# Autodesk Inventor assembly: ASY PNS 1600 Filter column D1000
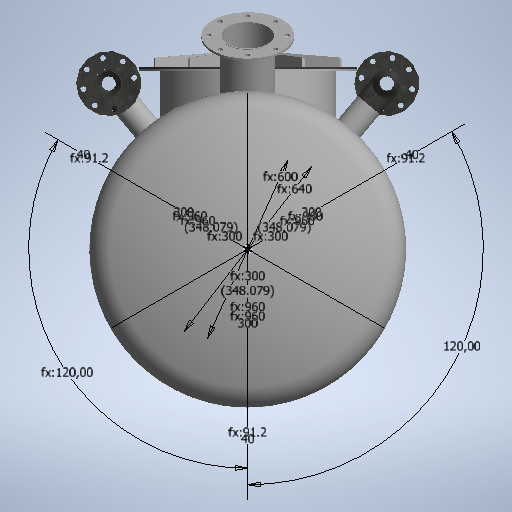
[picture p0: Inventor's stored thumbnail of the model, 512x512]
Saved by Autodesk Inventor 2025.1 (Build 291241020, 241B)
## iProperties
Created: 2025-02-13
Part Number: ASY PNS 1600 Filter column D1000
Document SubType Name: Assembly
Designer: pokla
Author: pokla
Revision Number: 3
## iProperties of the stored document MemberDocs/x3yapsqebEkdjevcwV0gr1zjvYf
Created: 2025-02-13
Part Number: ASY PNS 1600 Filter column D1000
Document SubType Name: Assembly
Designer: pokla
Author: pokla
Revision Number: 3
## iProperties of the stored document MemberDocs/xWb2o1nz5Ectr32dq2ydfqed0Rg
Created: 2025-02-13
Part Number: ASY PNS 1600 Filter column D1000
Document SubType Name: Assembly
Designer: pokla
Author: pokla
Revision Number: 3
## Documents named in this file (27)
- C:\Users\user\YandexDisk-badmisterfox\home pc\Inventor\PNS2-Panaevsk\Filter D1000\ASY PNS 1600 Filter column D1000.iam
- C:\Users\user\YandexDisk-badmisterfox\home pc\Inventor\PNS2-Panaevsk\Filter D1000\PNS-612 accses hatch flangeipt.ipt
- C:\Users\user\YandexDisk-badmisterfox\home pc\Inventor\PNS2-Panaevsk\Filter D1000\PNS 1601 DIM Filter column D1000.ipt
- C:\Users\user\YandexDisk-badmisterfox\home pc\Inventor\PNS2-Panaevsk\Filter D1000\PNS-611 accses hatch tube.ipt
- C:\Users\user\YandexDisk-badmisterfox\home pc\Inventor\PNS2-Panaevsk\Filter D1000\PNS-601 main tube D1000.ipt
- C:\Users\user\YandexDisk-badmisterfox\home pc\Inventor\PNS2-Panaevsk\Filter D1000\PNS- 652 tube.ipt
- C:\Users\user\YandexDisk-badmisterfox\home pc\Inventor\PNS2-Panaevsk\Filter D1000\PNS-633 charging blind flange.ipt
- C:\Users\user\YandexDisk-badmisterfox\home pc\Inventor\PNS2-Panaevsk\Filter D1000\PNS - 604 dished head D1000.ipt
- C:\Users\user\YandexDisk-badmisterfox\home pc\Inventor\PNS2-Panaevsk\Filter D1200\Fitting G1.ipt
- C:\Users\user\YandexDisk-badmisterfox\home pc\Inventor\PNS2-Panaevsk\Filter D1000\ASY PNS 1690 Filter legs D1000.iam
- C:\Users\user\YandexDisk-badmisterfox\home pc\Inventor\PNS2-Panaevsk\CC\en-US\DIN 2576 PN 10(2)\DIN 2576 Slip-On Flange for Welding Series 1 (ISO) - PN 10 80 x 88.9.ipt
- C:\Users\user\YandexDisk-badmisterfox\home pc\Inventor\PNS2-Panaevsk\Filter D1000\PNS 1633 charging blind flange.ipt
- C:\Users\user\YandexDisk-badmisterfox\home pc\Inventor\PNS2-Panaevsk\CC\en-US\DIN 2615-1 T\DIN 2615-1 Tee 88.9 x 5.6 S.ipt
- C:\Users\user\YandexDisk-badmisterfox\home pc\Inventor\PNS2-Panaevsk\CC\en-US\DIN 2616 CR (K)\DIN 2616 Concentric Reducer (K) 88.9 x 2.3 - 48.3 x 2.ipt
- C:\Users\user\YandexDisk-badmisterfox\home pc\Inventor\PNS2-Panaevsk\Filter D1000\ASY PNS 1610 charging hatch.iam
- C:\Users\user\YandexDisk-badmisterfox\home pc\Inventor\PNS2-Panaevsk\Filter D1000\PNS 1602 main Shell D1000.ipt
- C:\Users\user\YandexDisk-badmisterfox\home pc\Inventor\PNS2-Panaevsk\Filter D1000\PNS 1611 FDS tube 1.ipt
- C:\Users\user\YandexDisk-badmisterfox\home pc\Inventor\PNS2-Panaevsk\Filter D1000\PNS 1604 dished head D1000.ipt
- C:\Users\user\YandexDisk-badmisterfox\home pc\Inventor\PNS2-Panaevsk\CC\en-US\JIS B 2312 90 (2)\JIS B 2312 90 Deg Long Elbow Steel 80A x Sch 40.ipt
- C:\Users\user\YandexDisk-badmisterfox\home pc\Inventor\PNS2-Panaevsk\Filter D1000\filter-distribution-system 1000\ASY PNS 1650 filter-distribution-system 1000.iam
- C:\Users\user\YandexDisk-badmisterfox\home pc\Inventor\PNS2-Panaevsk\Filter D1000\PNS 1612 FDS tube 2.ipt
- C:\Users\user\YandexDisk-badmisterfox\home pc\Inventor\PNS2-Panaevsk\Filter D1000\PNS 1604 charging tube.ipt
- C:\Users\user\YandexDisk-badmisterfox\home pc\Inventor\PNS2-Panaevsk\Filter D1000\PNS 1606 charging flange round.ipt
- C:\Users\user\YandexDisk-badmisterfox\home pc\Inventor\PNS2-Panaevsk\Filter D1000\PNS 1607 charging flange cup.ipt
- C:\Users\user\YandexDisk-badmisterfox\home pc\Inventor\PNS2-Panaevsk\Filter D1000\PNS 1613 FDS tube 3.ipt
- C:\Users\user\YandexDisk-badmisterfox\home pc\Inventor\PNS2-Panaevsk\Filter D1000\PNS 1614 FDS tube 4.ipt
- C:\Users\user\YandexDisk-badmisterfox\home pc\Inventor\PNS2-Panaevsk\Filter D1000\PNS 1615 FDS tube 5.ipt
## Components (28 placed, 17 different names)
1. 000 DIM PNS600-Filter column D1200.ipt:1
2. PNS-612 accses hatch flangeipt.ipt:1 — Rigid:24, Rigid:25, Rigid:27, Rigid:28
3. PNS-611 accses hatch tube.ipt:1 — Rigid:10, Rigid:27
4. PNS-601 main tube D1000.ipt:1 — Rigid:10, Rigid:13, Rigid:14, Mate:1, Mate:2, Rigid:38, Rigid:39, Rigid:40
5. PNS- 652 tube.ipt:1 — Rigid:39, Rigid:41
6. PNS-612 accses hatch flangeipt.ipt:2 — Rigid:24, Rigid:26
7. PNS-633 charging blind flange.ipt:1
8. PNS- 652 tube.ipt:2 — Rigid:38, Rigid:44
9. PNS - 604 dished head D1200.ipt:1 — Rigid:13, Rigid:16
10. PNS - 604 dished head D1200.ipt:2 — Rigid:14, Rigid:15, Mate:3
11. Fitting G1.ipt:1 — Rigid:15
12. Fitting G1.ipt:2 — Rigid:16
13. PNS- 623 charging half tube.ipt:2 — Rigid:34, Rigid:40
14. PNS-633 charging blind flange.ipt:2
15. DIN 2576 Slip-On Flange for Welding Series 1 (ISO) - PN 10 500 x 508.ipt:1 — Rigid:28
16. PNS-612 accses hatch flangeipt.ipt:3 — Rigid:25, Rotational:5
17. PNS-612 accses hatch flangeipt.ipt:4 — Rigid:26
18. ASY PNS680-Filter legs D1200.iam:1 [sub-assembly] — Mate:4, Flush:2, Mate:5
19. PNS-733 charging flange round:1 — Rigid:34
20. DIN 2576 Slip-On Flange for Welding Series 1 (ISO) - PN 10 80 x 88.9:3
21. DIN 2615-1 Tee 88.9 x 5.6 S:1 — Rigid:41
22. Труба подключения фильтра D1200:4
23. DIN 2616 Concentric Reducer (K) 88.9 x 2.3 - 48.3 x 2:1
24. DIN 2576 Slip-On Flange for Welding Series 1 (ISO) - PN 10 80 x 88.9:4
25. DIN 2615-1 Tee 88.9 x 5.6 S:2 — Rigid:44
26. Труба подключения фильтра D1200:5
27. DIN 2616 Concentric Reducer (K) 88.9 x 2.3 - 48.3 x 2:2
28. ASY PNS-722 charging hatch:1 [sub-assembly] — Rotational:5
## Relationships (29: WeldJoint 20, Mate 5, RevoluteJoint 3, Flush 1)
- Rigid:10 [WeldJoint] (66 mm): PNS-611 accses hatch tube.ipt:1 ↔ PNS-601 main tube D1000.ipt:1
- Rigid:13 [WeldJoint]: PNS-601 main tube D1000.ipt:1 ↔ PNS - 604 dished head D1200.ipt:1
- Rigid:14 [WeldJoint]: PNS-601 main tube D1000.ipt:1 ↔ PNS - 604 dished head D1200.ipt:2
- Rigid:15 [WeldJoint]: PNS - 604 dished head D1200.ipt:2 ↔ Fitting G1.ipt:1
- Rigid:16 [WeldJoint]: PNS - 604 dished head D1200.ipt:1 ↔ Fitting G1.ipt:2
- Rigid:24 [WeldJoint]: PNS-612 accses hatch flangeipt.ipt:1 ↔ PNS-612 accses hatch flangeipt.ipt:2
- Rigid:25 [WeldJoint]: PNS-612 accses hatch flangeipt.ipt:1 ↔ PNS-612 accses hatch flangeipt.ipt:3
- Rigid:26 [WeldJoint]: PNS-612 accses hatch flangeipt.ipt:2 ↔ PNS-612 accses hatch flangeipt.ipt:4
- Rigid:27 [WeldJoint]: PNS-612 accses hatch flangeipt.ipt:1 ↔ PNS-611 accses hatch tube.ipt:1
- Rigid:28 [WeldJoint]: PNS-612 accses hatch flangeipt.ipt:1 ↔ DIN 2576 Slip-On Flange for Welding Series 1 (ISO) - PN 10 500 x 508.ipt:1
- Mate:1: PNS-601 main tube D1000.ipt:1
- Mate:2: PNS-601 main tube D1000.ipt:1
- Mate:3 (2615 mm): PNS - 604 dished head D1200.ipt:2
- Mate:4: ASY PNS680-Filter legs D1200.iam:1
- Flush:2: ASY PNS680-Filter legs D1200.iam:1
- Mate:5: ASY PNS680-Filter legs D1200.iam:1
- Rigid:34 [WeldJoint]: PNS- 623 charging half tube.ipt:2 ↔ PNS-733 charging flange round:1
- [RevoluteJoint]: DIN 2615-1 Tee 88.9 x 5.6 S:1 ↔ Труба подключения фильтра D1200:4
- [WeldJoint]: DIN 2576 Slip-On Flange for Welding Series 1 (ISO) - PN 10 80 x 88.9:3 ↔ Труба подключения фильтра D1200:4
- [WeldJoint]: DIN 2615-1 Tee 88.9 x 5.6 S:1 ↔ DIN 2616 Concentric Reducer (K) 88.9 x 2.3 - 48.3 x 2:1
- Rigid:38 [WeldJoint]: PNS-601 main tube D1000.ipt:1 ↔ PNS- 652 tube.ipt:2
- Rigid:39 [WeldJoint]: PNS-601 main tube D1000.ipt:1 ↔ PNS- 652 tube.ipt:1
- Rigid:40 [WeldJoint]: PNS-601 main tube D1000.ipt:1 ↔ PNS- 623 charging half tube.ipt:2
- Rigid:41 [WeldJoint]: PNS- 652 tube.ipt:1 ↔ DIN 2615-1 Tee 88.9 x 5.6 S:1
- [RevoluteJoint]: DIN 2615-1 Tee 88.9 x 5.6 S:2 ↔ Труба подключения фильтра D1200:5
- [WeldJoint]: DIN 2576 Slip-On Flange for Welding Series 1 (ISO) - PN 10 80 x 88.9:4 ↔ Труба подключения фильтра D1200:5
- [WeldJoint]: DIN 2615-1 Tee 88.9 x 5.6 S:2 ↔ DIN 2616 Concentric Reducer (K) 88.9 x 2.3 - 48.3 x 2:2
- Rigid:44 [WeldJoint]: PNS- 652 tube.ipt:2 ↔ DIN 2615-1 Tee 88.9 x 5.6 S:2
- Rotational:5 [RevoluteJoint]: PNS-612 accses hatch flangeipt.ipt:3 ↔ ASY PNS-722 charging hatch:1
## Named parameters: d74_d69 = 0 mm, d75_d70 = 175 deg, d76_d71 = 0 mm, d77_d72 = 0 mm, d64_d74_d69 = 0 mm, d65_d75_d70 = -5 deg, d66_d76_d71 = 0 mm, d67_d77_d72 = 0 mm
